# Autodesk Inventor assembly: 50T nanotube cluster no 14T
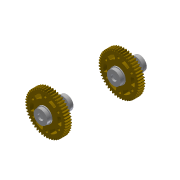
[picture p0: Inventor's stored thumbnail of the model, 180x180]
Saved by Autodesk Inventor 2013 (Build 170138000, 138)
## iProperties
Created: 2013-09-01
Part Number: 50T nanotube cluster no 14T
Document SubType Name: Assembly
Designer: Nemo
Mass: 97.888 g
Surface Area: 167.806 cm^2
Volume: 32.0625 cm^3
Density: 3.05303 g/cm^3
Author: Nemo
## Documents named in this file (4)
- H:\Nemo\Documents\Robotics\COTS Parts\Gearboxes\Components\50T nanotube cluster no 14T.iam
- H:\Nemo\Documents\Robotics\COTS Parts\Gears - VexPro\Gear 20dp 375hex 50T Vex.ipt
- H:\Nemo\Documents\Robotics\COTS Parts\Bearings - VexPro\Flanged Bearing - 0.375in Round ID x 0.875in OD.ipt
- H:\Nemo\Documents\Robotics\COTS Parts\Gearboxes\Components\VexPro Double Reduction Components\VexBox cluster shaft.ipt
## Components (4 placed, 3 different names)
1. Gear 20dp 375hex 50T Vex:1 — Mate:3, Mate:5, Angle:1
2. Flanged Bearing - 0.375in Round ID x 0.875in OD:1 — Mate:2, Mate:5
3. VexBox cluster shaft:1 — Mate:1, Mate:3, Mate:4, Angle:1
4. Flanged Bearing - 0.375in Round ID x 0.875in OD:2 — Mate:1, Mate:2, Mate:4
## Relationships (6: Mate 5, Angle 1)
- Mate:1: VexBox cluster shaft:1 ↔ Flanged Bearing - 0.375in Round ID x 0.875in OD:2
- Mate:2 (-31.75 mm): Flanged Bearing - 0.375in Round ID x 0.875in OD:1 ↔ Flanged Bearing - 0.375in Round ID x 0.875in OD:2
- Mate:3: Gear 20dp 375hex 50T Vex:1 ↔ VexBox cluster shaft:1
- Mate:4 (0.254 mm): VexBox cluster shaft:1 ↔ Flanged Bearing - 0.375in Round ID x 0.875in OD:2
- Mate:5 (0.254 mm): Gear 20dp 375hex 50T Vex:1 ↔ Flanged Bearing - 0.375in Round ID x 0.875in OD:1
- Angle:1 (0 deg): Gear 20dp 375hex 50T Vex:1 ↔ VexBox cluster shaft:1
